# Autodesk Inventor assembly: tc_switchplate
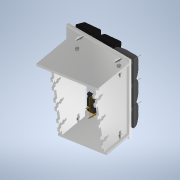
[picture p0: Inventor's stored thumbnail of the model, 180x180]
Saved by Autodesk Inventor 2020.1 (Build 241239000, 239)
## iProperties
Created: 2019-07-07
Part Number: tc_switchplate
Document SubType Name: Assembly
Designer: Thibault
Author: Thibault
## Documents named in this file (10)
- C:\Users\Thibault Polge\Documents\Habilis\mech\tc_switchplate.iam
- C:\Users\Thibault Polge\Documents\Habilis\mech\tc_base_plate.ipt
- C:\Users\Thibault Polge\Documents\Habilis\mech\mx\TC-R1 2×1 A.iam
- C:\Users\Thibault Polge\Documents\Habilis\mech\mx\TC-R1 2×1 B.iam
- C:\Users\Thibault Polge\Documents\Habilis\mech\mx.iam
- C:\Users\Thibault Polge\Documents\Habilis\mech\tc_support_front.ipt
- C:\Users\Thibault Polge\Documents\Habilis\mech\tc_support_down.ipt
- C:\Users\Thibault Polge\Documents\Inventor\Content Center Files\R2020\fr-FR\BS 4168(1)\BS 4168 - M1,6 x 8(1).ipt
- C:\Users\Thibault Polge\Documents\Habilis\mech\mx\DSA-1x1.iam
- C:\Users\Thibault Polge\Documents\Habilis\mech\tc_support_back.ipt
## Components (19 placed, 8 different names)
1. tc_base_plate:1 — Placage:1, Placage:2, Placage:3, Placage:4, Placage:5, Placage:6, Placage:7, Affleurement:1, Placage:8, Placage:9, Placage:10, Affleurement:2, Placage:11, Placage:12, Placage:13, Placage:14, Placage:15, Placage:16, Affleurement:3, Placage:17, Placage:18, Affleurement:4, Affleurement:5, Affleurement:6, Logement:3, Logement:4, Affleurement:9, Placage:23, Placage:24, Logement:5, Logement:6
2. DSA-1x1:1 [sub-assembly] — Placage:4, Placage:9, Placage:15
3. DSA-1x1:2 [sub-assembly] — Placage:2, Affleurement:1, Placage:12
4. DSA-1x1:3 [sub-assembly] — Placage:5, Placage:10, Placage:16
5. TC-R1 2×1 A:4 [sub-assembly] — Placage:3, Placage:7, Placage:13
6. TC-R1 2×1 B:5 [sub-assembly] — Placage:6, Affleurement:2, Placage:14
7. DSA-1x1:6 [sub-assembly] — Placage:1, Placage:8, Placage:11
8. tc_support_front:1 — Affleurement:3, Placage:17, Placage:18, Logement:1, Logement:2, Affleurement:11, Placage:27, Placage:28
9. tc_support_down:1 — Affleurement:11, Placage:27, Placage:28
10. tc_support_down:2 — Affleurement:10, Placage:25, Placage:26
11. BS 4168 : Pièce 1 Vis cylindrique à six pans creux - Métrique M1,6 x 8:1 — Logement:1
12. BS 4168 : Pièce 1 Vis cylindrique à six pans creux - Métrique M1,6 x 8:2 — Logement:2
13. BS 4168 : Pièce 1 Vis cylindrique à six pans creux - Métrique M1,6 x 8:3 — Logement:3
14. BS 4168 : Pièce 1 Vis cylindrique à six pans creux - Métrique M1,6 x 8:4 — Logement:4
15. tc_support_back:1 — Affleurement:9, Placage:23, Placage:24, Logement:7, Logement:8, Affleurement:10, Placage:25, Placage:26
16. BS 4168 : Pièce 1 Vis cylindrique à six pans creux - Métrique M1,6 x 8:5 — Logement:5
17. BS 4168 : Pièce 1 Vis cylindrique à six pans creux - Métrique M1,6 x 8:6 — Logement:6
18. BS 4168 : Pièce 1 Vis cylindrique à six pans creux - Métrique M1,6 x 8:7 — Logement:7
19. BS 4168 : Pièce 1 Vis cylindrique à six pans creux - Métrique M1,6 x 8:8 — Logement:8
## Relationships (41: Mate 24, Flush 9, Insert 8)
- Placage:1 [Mate]: tc_base_plate:1 ↔ DSA-1x1:6
- Placage:2 [Mate]: tc_base_plate:1 ↔ DSA-1x1:2
- Placage:3 [Mate]: tc_base_plate:1 ↔ TC-R1 2×1 A:4
- Placage:4 [Mate]: tc_base_plate:1 ↔ DSA-1x1:1
- Placage:5 [Mate]: tc_base_plate:1 ↔ DSA-1x1:3
- Placage:6 [Mate]: tc_base_plate:1 ↔ TC-R1 2×1 B:5
- Placage:7 [Mate]: tc_base_plate:1 ↔ TC-R1 2×1 A:4
- Affleurement:1 [Flush]: tc_base_plate:1 ↔ DSA-1x1:2
- Placage:8 [Mate]: tc_base_plate:1 ↔ DSA-1x1:6
- Placage:9 [Mate]: tc_base_plate:1 ↔ DSA-1x1:1
- Placage:10 [Mate]: tc_base_plate:1 ↔ DSA-1x1:3
- Affleurement:2 [Flush]: tc_base_plate:1 ↔ TC-R1 2×1 B:5
- Placage:11 [Mate]: tc_base_plate:1 ↔ DSA-1x1:6
- Placage:12 [Mate]: tc_base_plate:1 ↔ DSA-1x1:2
- Placage:13 [Mate]: tc_base_plate:1 ↔ TC-R1 2×1 A:4
- Placage:14 [Mate]: tc_base_plate:1 ↔ TC-R1 2×1 B:5
- Placage:15 [Mate]: tc_base_plate:1 ↔ DSA-1x1:1
- Placage:16 [Mate]: tc_base_plate:1 ↔ DSA-1x1:3
- Affleurement:3 [Flush]: tc_base_plate:1 ↔ tc_support_front:1
- Placage:17 [Mate]: tc_base_plate:1 ↔ tc_support_front:1
- Placage:18 [Mate]: tc_base_plate:1 ↔ tc_support_front:1
- Affleurement:4 [Flush]: tc_base_plate:1
- Affleurement:5 [Flush]: tc_base_plate:1
- Affleurement:6 [Flush]: tc_base_plate:1
- Logement:1 [Insert]: tc_support_front:1 ↔ BS 4168 : Pièce 1 Vis cylindrique à six pans creux - Métrique M1,6 x 8:1
- Logement:2 [Insert]: tc_support_front:1 ↔ BS 4168 : Pièce 1 Vis cylindrique à six pans creux - Métrique M1,6 x 8:2
- Logement:3 [Insert]: tc_base_plate:1 ↔ BS 4168 : Pièce 1 Vis cylindrique à six pans creux - Métrique M1,6 x 8:3
- Logement:4 [Insert]: tc_base_plate:1 ↔ BS 4168 : Pièce 1 Vis cylindrique à six pans creux - Métrique M1,6 x 8:4
- Affleurement:9 [Flush]: tc_base_plate:1 ↔ tc_support_back:1
- Placage:23 [Mate]: tc_base_plate:1 ↔ tc_support_back:1
- Placage:24 [Mate]: tc_base_plate:1 ↔ tc_support_back:1
- Logement:5 [Insert]: tc_base_plate:1 ↔ BS 4168 : Pièce 1 Vis cylindrique à six pans creux - Métrique M1,6 x 8:5
- Logement:6 [Insert]: tc_base_plate:1 ↔ BS 4168 : Pièce 1 Vis cylindrique à six pans creux - Métrique M1,6 x 8:6
- Logement:7 [Insert]: tc_support_back:1 ↔ BS 4168 : Pièce 1 Vis cylindrique à six pans creux - Métrique M1,6 x 8:7
- Logement:8 [Insert]: tc_support_back:1 ↔ BS 4168 : Pièce 1 Vis cylindrique à six pans creux - Métrique M1,6 x 8:8
- Affleurement:10 [Flush]: tc_support_down:2 ↔ tc_support_back:1
- Placage:25 [Mate]: tc_support_down:2 ↔ tc_support_back:1
- Placage:26 [Mate]: tc_support_down:2 ↔ tc_support_back:1
- Affleurement:11 [Flush]: tc_support_front:1 ↔ tc_support_down:1
- Placage:27 [Mate]: tc_support_front:1 ↔ tc_support_down:1
- Placage:28 [Mate]: tc_support_front:1 ↔ tc_support_down:1
